# Autodesk Inventor assembly: Potencia
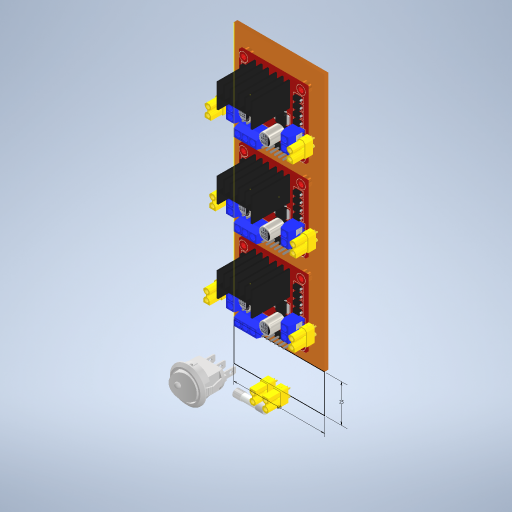
[picture p0: Inventor's stored thumbnail of the model, 512x512]
Saved by Autodesk Inventor 2024.2 (Build 282272000, 272)
## iProperties
Created: 2024-08-03
Part Number: Potencia
Document SubType Name: Assembly
Designer: Admin
Author: Admin
## Documents named in this file (6)
- C:\Users\Admin\Documents\GitHub\ExplorateurErrant\Potencia.iam
- C:\Users\Admin\Documents\GitHub\ExplorateurErrant\Potencia\BasePotencia.ipt
- C:\Users\Admin\Documents\GitHub\ExplorateurErrant\Potencia\H-Bridge\H-brug.ipt
- C:\Users\Admin\Documents\GitHub\ExplorateurErrant\Potencia\XT30-Female\XT30Female.ipt
- C:\Users\Admin\Documents\GitHub\ExplorateurErrant\Potencia\SwitchKCD\KCD1\KCD1.ipt
- C:\Users\Admin\Documents\GitHub\ExplorateurErrant\Potencia\Fuse\EuropeanFuse3A.ipt
## Components (14 placed, 5 different names)
1. BasePotencia:1 — Mate:1, Mate:2, Mate:3, Mate:4, Mate:5, Mate:6, Mate:7, Mate:8, Mate:9
2. H-brug:1 — Mate:1, Mate:2, Mate:3
3. H-brug:2 — Mate:4, Mate:5, Mate:6
4. H-brug:3 — Mate:7, Mate:8, Mate:9
5. XT30Female:1
6. XT30Female:2
7. XT30Female:3
8. XT30Female:4
9. XT30Female:5
10. XT30Female:6
11. KCD1:1
12. XT30Female:7
13. XT30Female:8
14. EuropeanFuse3A:1
## Relationships (9: Mate 9)
- Mate:1: BasePotencia:1 ↔ H-brug:1
- Mate:2: BasePotencia:1 ↔ H-brug:1
- Mate:3: BasePotencia:1 ↔ H-brug:1
- Mate:4: BasePotencia:1 ↔ H-brug:2
- Mate:5: BasePotencia:1 ↔ H-brug:2
- Mate:6: BasePotencia:1 ↔ H-brug:2
- Mate:7: BasePotencia:1 ↔ H-brug:3
- Mate:8: BasePotencia:1 ↔ H-brug:3
- Mate:9: BasePotencia:1 ↔ H-brug:3
